# Autodesk Inventor assembly: MONTAGEM TCC
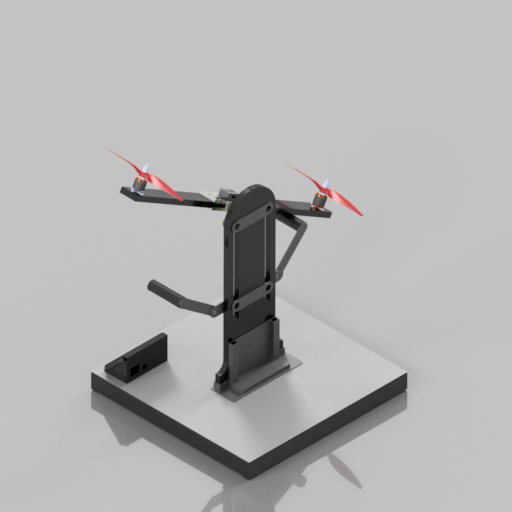
[picture p0: Inventor's stored thumbnail of the model, 512x512]
Saved by Autodesk Inventor 2025.2 (Build 292293000, 293)
## iProperties
Created: 2024-04-26
Part Number: MONTAGEM TCC
Document SubType Name: Assembly
Designer: phmca
Author: phmca
## Documents named in this file (24)
- C:\Users\phmca\OneDrive\Documentos\TCC\TCC\MONTAGEM TCC.iam
- C:\Users\phmca\OneDrive\Documentos\TCC\TCC\Chapa - Inox.ipt
- C:\Users\phmca\OneDrive\Documentos\TCC\TCC\Painel Vertical.ipt
- C:\Users\phmca\OneDrive\Documentos\TCC\TCC\Ripas - Base - 458 mm.ipt
- C:\Users\phmca\OneDrive\Documentos\TCC\TCC\Ripas - Base - 500 mm.ipt
- C:\Users\phmca\OneDrive\Documentos\TCC\TCC\Ripas - Base - 200 mm.ipt
- C:\Users\phmca\OneDrive\Documentos\TCC\TCC\AIS2023\SKF_UCFL 205.iam
- C:\Users\phmca\OneDrive\Documentos\TCC\TCC\Junta.ipt
- C:\Users\phmca\OneDrive\Documentos\TCC\TCC\Pás.ipt
- C:\Users\phmca\OneDrive\Documentos\TCC\TCC\Chapa - aperto do rolamento.ipt
- C:\Users\phmca\OneDrive\Documentos\TCC\TCC\Suporte batente.ipt
- C:\Users\phmca\OneDrive\Documentos\TCC\TCC\Batente.ipt
- C:\Users\phmca\OneDrive\Documentos\TCC\TCC\Cantoneira Esquerda.ipt
- C:\Users\phmca\OneDrive\Documentos\TCC\TCC\Cantoneira Esquerda_MIR.ipt
- C:\Users\phmca\OneDrive\Documentos\TCC\TCC\Base cantoneiras.ipt
- C:\Users\phmca\OneDrive\Documentos\TCC\TCC\Continuação canaleta.ipt
- C:\Users\phmca\OneDrive\Documentos\TCC\TCC\Continuação canaleta_MIR.ipt
- C:\Users\phmca\OneDrive\Documentos\TCC\TCC\brushless-motor-with-prop-1.snapshot.1\assembly\assembly.iam
- C:\Users\phmca\OneDrive\Documentos\TCC\TCC\Case MPU.ipt
- C:\Users\phmca\OneDrive\Documentos\TCC\TCC\MPU_6050 v1.iam
- C:\Users\phmca\OneDrive\Área de Trabalho\CASE - IHM.ipt
- C:\Users\phmca\OneDrive\Área de Trabalho\CASE - IHM V2.ipt
- C:\Users\phmca\Downloads\nextion-3-5-hmi-nx4832t035-1.snapshot.7\Nextion 3.5 inch HMI (NX4832T035)\Nextion_3.5_HMI_NX4832T035\Nextion_3.5_HMI_NX4832T035\Nextion_3.5_HMI_NX4832T035.ipt
- C:\Users\phmca\OneDrive\Área de Trabalho\caneta_duo.ipt
## Components (34 placed, 23 different names)
1. Chapa - Inox:1 — Alinhado:14, Alinhado:15, Coincidente:7, Coincidente:26, Coincidente:57, Coincidente:60, Coincidente:63, Alinhado:22, Alinhado:23
2. Painel Vertical:1 — Alinhado:9, Coincidente:3, Coincidente:5, Alinhado:13, Rotativa:1, Rotativa:2, Rotativa:4, Coincidente:13, Coincidente:15, Coincidente:16, Coincidente:22, Coincidente:23, Coincidente:24, Coincidente:25, Coincidente:27, Coincidente:31, Coincidente:33, Ângulo:7, Coincidente:35, Coincidente:36, Coincidente:37, Coincidente:40, Coincidente:43, Coincidente:46, Coincidente:61, Coincidente:62
3. Ripas - Base - 458 mm:1 — Rígida:3, Alinhado:1, Alinhado:15
4. Ripas - Base - 500 mm:1 — Rígida:2, Rígida:3, Coincidente:1, Coincidente:2, Alinhado:7
5. Ripas - Base - 500 mm:2 — Rígida:1, Alinhado:3, Alinhado:6, Alinhado:8, Alinhado:14, Coincidente:7, Coincidente:58
6. Ripas - Base - 458 mm:2 — Rígida:1, Rígida:2, Alinhado:4, Coincidente:59
7. Ripas - Base - 458 mm:3 — Alinhado:2, Alinhado:3, Coincidente:1
8. Ripas - Base - 458 mm:4 — Alinhado:5, Alinhado:6, Coincidente:2, Alinhado:9, Coincidente:3, Coincidente:4, Alinhado:11
9. Ripas - Base - 200 mm:1 — Coincidente:6, Alinhado:12, Alinhado:13
10. Ripas - Base - 200 mm:2 — Alinhado:10, Coincidente:4, Alinhado:11, Coincidente:5
11. SKF_UCFL 205:1 [sub-assembly] — Rotativa:1, Rotativa:2, Rotativa:3
12. Junta:1 — Rotativa:3, Coincidente:8, Coincidente:9, Alinhado:16, Coincidente:10, Coincidente:11, Alinhado:17, Rotativa:7, Alinhado:21
13. Pás:1 — Coincidente:10, Coincidente:11, Alinhado:17, Coincidente:47, Ângulo:9, Coincidente:49, Coincidente:50, Ângulo:10, Tangente:1, Tangente:2
14. Pás:2 — Coincidente:8, Coincidente:9, Alinhado:16, Coincidente:51, Ângulo:11, Coincidente:52, Ângulo:12, Coincidente:54
15. Chapa - aperto do rolamento:1 — Rotativa:4, Coincidente:31
16. Suporte batente:1 — Coincidente:13, Rotativa:5, Coincidente:14, Ângulo:1, Rotativa:6, Coincidente:17, Ângulo:2, Coincidente:18, Ângulo:3, Rotativa:8
17. Batente:1 — Rotativa:5, Tangente:1, Rotativa:8, Tangente:2
18. Batente:2 — Rotativa:6
19. Chapa - aperto do rolamento:2 — Coincidente:16, Coincidente:19, Ângulo:4, Coincidente:20, Ângulo:5
20. Cantoneira Esquerda:1 — Coincidente:22, Coincidente:23, Alinhado:19, Coincidente:28, Coincidente:29, Coincidente:30, Coincidente:35, Coincidente:38, Ângulo:8, Coincidente:41, Coincidente:42
21. Cantoneira Esquerda_MIR:1 — Coincidente:24, Coincidente:25, Alinhado:19, Coincidente:44, Coincidente:45
22. Base cantoneiras:1 — Coincidente:26, Coincidente:27, Coincidente:28, Coincidente:29, Coincidente:30, Coincidente:36, Coincidente:37, Coincidente:46
23. Continuação canaleta:1 — Coincidente:40, Coincidente:41, Coincidente:42
24. Continuação canaleta_MIR:1 — Coincidente:43, Coincidente:44, Coincidente:45, Coincidente:56
25. assembly:1 [sub-assembly] — Coincidente:48, Coincidente:49, Alinhado:20
26. assembly:2 [sub-assembly] — Coincidente:53, Coincidente:54, Coincidente:55
27. Case MPU:1 — Rotativa:7, Alinhado:21, Rotativa:9
28. MPU_6050 v1:1 [sub-assembly] — Rotativa:9
29. Base cantoneiras:2 — Coincidente:56
30. CASE - IHM:1 — Coincidente:57, Coincidente:58, Coincidente:59
31. Base cantoneiras:3 — Coincidente:60, Coincidente:61, Coincidente:62
32. CASE - IHM V2:1 — Coincidente:63, Alinhado:22, Alinhado:23, Rotativa:10, Rotativa:11
33. Nextion_3.5_HMI_NX4832T035:1 — Rotativa:10
34. caneta_duo:1 — Rotativa:11
## Relationships (110: Mate 60, Flush 23, RevoluteJoint 11, Angle 11, WeldJoint 3, Tangent 2)
- Rígida:1 [WeldJoint]: Ripas - Base - 500 mm:2 ↔ Ripas - Base - 458 mm:2
- Rígida:2 [WeldJoint]: Ripas - Base - 500 mm:1 ↔ Ripas - Base - 458 mm:2
- Rígida:3 [WeldJoint]: Ripas - Base - 458 mm:1 ↔ Ripas - Base - 500 mm:1
- Alinhado:1 [Flush] (129 mm): Ripas - Base - 458 mm:1
- Alinhado:2 [Flush]: Ripas - Base - 458 mm:3
- Alinhado:3 [Flush]: Ripas - Base - 500 mm:2 ↔ Ripas - Base - 458 mm:3
- Coincidente:1 [Mate]: Ripas - Base - 500 mm:1 ↔ Ripas - Base - 458 mm:3
- Alinhado:4 [Flush] (129 mm): Ripas - Base - 458 mm:2
- Alinhado:5 [Flush]: Ripas - Base - 458 mm:4
- Alinhado:6 [Flush]: Ripas - Base - 500 mm:2 ↔ Ripas - Base - 458 mm:4
- Coincidente:2 [Mate]: Ripas - Base - 500 mm:1 ↔ Ripas - Base - 458 mm:4
- Alinhado:7 [Flush] (221.5 mm): Ripas - Base - 500 mm:1
- Alinhado:8 [Flush] (221.5 mm): Ripas - Base - 500 mm:2
- Alinhado:9 [Flush]: Painel Vertical:1 ↔ Ripas - Base - 458 mm:4
- Coincidente:3 [Mate]: Painel Vertical:1 ↔ Ripas - Base - 458 mm:4
- Alinhado:10 [Flush]: Ripas - Base - 200 mm:2
- Coincidente:4 [Mate]: Ripas - Base - 458 mm:4 ↔ Ripas - Base - 200 mm:2
- Alinhado:11 [Flush]: Ripas - Base - 458 mm:4 ↔ Ripas - Base - 200 mm:2
- Coincidente:5 [Mate]: Painel Vertical:1 ↔ Ripas - Base - 200 mm:2
- Coincidente:6 [Mate]: Ripas - Base - 200 mm:1
- Alinhado:12 [Flush]: Ripas - Base - 200 mm:1
- Alinhado:13 [Flush]: Painel Vertical:1 ↔ Ripas - Base - 200 mm:1
- Alinhado:14 [Flush]: Chapa - Inox:1 ↔ Ripas - Base - 500 mm:2
- Alinhado:15 [Flush]: Chapa - Inox:1 ↔ Ripas - Base - 458 mm:1
- Coincidente:7 [Mate]: Chapa - Inox:1 ↔ Ripas - Base - 500 mm:2
- Rotativa:1 [RevoluteJoint]: Painel Vertical:1 ↔ SKF_UCFL 205:1
- Rotativa:2 [RevoluteJoint]: Painel Vertical:1 ↔ SKF_UCFL 205:1
- Rotativa:3 [RevoluteJoint]: SKF_UCFL 205:1 ↔ Junta:1
- Coincidente:8 [Mate]: Junta:1 ↔ Pás:2
- Coincidente:9 [Mate]: Junta:1 ↔ Pás:2
- Alinhado:16 [Flush]: Junta:1 ↔ Pás:2
- Coincidente:10 [Mate]: Junta:1 ↔ Pás:1
- Coincidente:11 [Mate]: Junta:1 ↔ Pás:1
- Alinhado:17 [Flush]: Junta:1 ↔ Pás:1
- Rotativa:4 [RevoluteJoint]: Painel Vertical:1 ↔ Chapa - aperto do rolamento:1
- Coincidente:13 [Mate]: Painel Vertical:1 ↔ Suporte batente:1
- Rotativa:5 [RevoluteJoint]: Suporte batente:1 ↔ Batente:1
- Coincidente:14 [Mate]: Suporte batente:1
- Ângulo:1 [Angle] (0 deg): Suporte batente:1
- Coincidente:15 [Mate]: Painel Vertical:1
- Rotativa:6 [RevoluteJoint]: Suporte batente:1 ↔ Batente:2
- Coincidente:16 [Mate]: Painel Vertical:1 ↔ Chapa - aperto do rolamento:2
- Coincidente:17 [Mate]: Suporte batente:1
- Ângulo:2 [Angle] (0 deg): Suporte batente:1
- Coincidente:18 [Mate]: Suporte batente:1
- Ângulo:3 [Angle] (0 deg): Suporte batente:1
- Coincidente:19 [Mate]: Chapa - aperto do rolamento:2
- Ângulo:4 [Angle] (0 deg): Chapa - aperto do rolamento:2
- Coincidente:20 [Mate]: Chapa - aperto do rolamento:2
- Ângulo:5 [Angle] (0 deg): Chapa - aperto do rolamento:2
- Coincidente:21 [Mate]
- Alinhado:18 [Flush]
- Coincidente:22 [Mate]: Painel Vertical:1 ↔ Cantoneira Esquerda:1
- Coincidente:23 [Mate]: Painel Vertical:1 ↔ Cantoneira Esquerda:1
- Coincidente:24 [Mate]: Painel Vertical:1 ↔ Cantoneira Esquerda_MIR:1
- Coincidente:25 [Mate]: Painel Vertical:1 ↔ Cantoneira Esquerda_MIR:1
- Alinhado:19 [Flush]: Cantoneira Esquerda:1 ↔ Cantoneira Esquerda_MIR:1
- Coincidente:26 [Mate]: Chapa - Inox:1 ↔ Base cantoneiras:1
- Coincidente:27 [Mate]: Painel Vertical:1 ↔ Base cantoneiras:1
- Coincidente:28 [Mate]: Cantoneira Esquerda:1 ↔ Base cantoneiras:1
- Coincidente:29 [Mate]: Cantoneira Esquerda:1 ↔ Base cantoneiras:1
- Coincidente:30 [Mate]: Cantoneira Esquerda:1 ↔ Base cantoneiras:1
- Coincidente:31 [Mate]: Painel Vertical:1 ↔ Chapa - aperto do rolamento:1
- Coincidente:33 [Mate]: Painel Vertical:1
- Ângulo:7 [Angle] (0 deg): Painel Vertical:1
- Coincidente:35 [Mate]: Painel Vertical:1 ↔ Cantoneira Esquerda:1
- Coincidente:36 [Mate]: Painel Vertical:1 ↔ Base cantoneiras:1
- Coincidente:37 [Mate]: Painel Vertical:1 ↔ Base cantoneiras:1
- Coincidente:38 [Mate]: Cantoneira Esquerda:1
- Ângulo:8 [Angle] (0 deg): Cantoneira Esquerda:1
- Coincidente:39 [Mate]
- Coincidente:40 [Mate]: Painel Vertical:1 ↔ Continuação canaleta:1
- Coincidente:41 [Mate]: Cantoneira Esquerda:1 ↔ Continuação canaleta:1
- Coincidente:42 [Mate]: Cantoneira Esquerda:1 ↔ Continuação canaleta:1
- Coincidente:43 [Mate]: Painel Vertical:1 ↔ Continuação canaleta_MIR:1
- Coincidente:44 [Mate]: Cantoneira Esquerda_MIR:1 ↔ Continuação canaleta_MIR:1
- Coincidente:45 [Mate]: Cantoneira Esquerda_MIR:1 ↔ Continuação canaleta_MIR:1
- Coincidente:46 [Mate]: Painel Vertical:1 ↔ Base cantoneiras:1
- Coincidente:47 [Mate]: Pás:1
- Ângulo:9 [Angle] (0 deg): Pás:1
- Coincidente:48 [Mate]: assembly:1
- Coincidente:49 [Mate]: Pás:1 ↔ assembly:1
- Coincidente:50 [Mate]: Pás:1
- Ângulo:10 [Angle] (0 deg): Pás:1
- Alinhado:20 [Flush]: assembly:1
- Coincidente:51 [Mate]: Pás:2
- Ângulo:11 [Angle] (0 deg): Pás:2
- Coincidente:52 [Mate]: Pás:2
- Ângulo:12 [Angle] (0 deg): Pás:2
- Coincidente:53 [Mate]: assembly:2
- Coincidente:54 [Mate]: Pás:2 ↔ assembly:2
- Coincidente:55 [Mate]: assembly:2
- Tangente:1: Pás:1 ↔ Batente:1
- Rotativa:7 [RevoluteJoint]: Junta:1 ↔ Case MPU:1
- Alinhado:21 [Flush]: Junta:1 ↔ Case MPU:1
- Rotativa:8 [RevoluteJoint]: Suporte batente:1 ↔ Batente:1
- Tangente:2: Pás:1 ↔ Batente:1
- Rotativa:9 [RevoluteJoint]: Case MPU:1 ↔ MPU_6050 v1:1
- Coincidente:56 [Mate]: Continuação canaleta_MIR:1 ↔ Base cantoneiras:2
- Coincidente:57 [Mate]: Chapa - Inox:1 ↔ CASE - IHM:1
- Coincidente:58 [Mate]: Ripas - Base - 500 mm:2 ↔ CASE - IHM:1
- Coincidente:59 [Mate]: Ripas - Base - 458 mm:2 ↔ CASE - IHM:1
- Coincidente:60 [Mate]: Chapa - Inox:1 ↔ Base cantoneiras:3
- Coincidente:61 [Mate] (0.5 mm): Painel Vertical:1 ↔ Base cantoneiras:3
- Coincidente:62 [Mate] (1 mm): Painel Vertical:1 ↔ Base cantoneiras:3
- Coincidente:63 [Mate]: Chapa - Inox:1 ↔ CASE - IHM V2:1
- Alinhado:22 [Flush]: Chapa - Inox:1 ↔ CASE - IHM V2:1
- Alinhado:23 [Flush]: Chapa - Inox:1 ↔ CASE - IHM V2:1
- Rotativa:10 [RevoluteJoint]: CASE - IHM V2:1 ↔ Nextion_3.5_HMI_NX4832T035:1
- Rotativa:11 [RevoluteJoint]: CASE - IHM V2:1 ↔ caneta_duo:1
